# Autodesk Inventor assembly: PBotCatapult
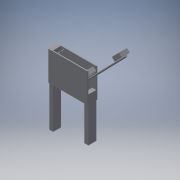
[picture p0: Inventor's stored thumbnail of the model, 180x180]
Saved by Autodesk Inventor 2018 (Build 220112000, 112)
## iProperties
Created: 2018-05-31
Part Number: PBotCatapult
Document SubType Name: Assembly
Designer: choices
Author: choices
## Documents named in this file (5)
- C:\Users\choices\Documents\PBotCatapult.iam
- C:\Users\choices\Documents\PBotArm.ipt
- C:\Users\choices\Documents\PBotCatapultShell.ipt
- C:\Users\choices\Documents\SolenoidArm.ipt
- C:\Users\choices\Documents\SolenoidCase.ipt
## Components (4 placed, 4 different names)
1. PBotArm:1 — Mate:1, Mate:2, Mate:7
2. PBotCatapultShell:1 — Mate:1, Mate:2, Mate:5, Mate:6
3. SolenoidArm:1 — Mate:3, Mate:4, Mate:7
4. SolenoidCase:1 — Mate:3, Mate:4, Mate:5, Mate:6
## Relationships (7: Mate 7)
- Mate:1: PBotArm:1 ↔ PBotCatapultShell:1
- Mate:2 (50.8 mm): PBotArm:1 ↔ PBotCatapultShell:1
- Mate:3: SolenoidArm:1 ↔ SolenoidCase:1
- Mate:4: SolenoidArm:1 ↔ SolenoidCase:1
- Mate:5: PBotCatapultShell:1 ↔ SolenoidCase:1
- Mate:6 (44.45 mm): PBotCatapultShell:1 ↔ SolenoidCase:1
- Mate:7: PBotArm:1 ↔ SolenoidArm:1
